# Autodesk Inventor assembly: Tensioner
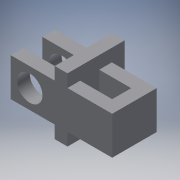
[picture p0: Inventor's stored thumbnail of the model, 180x180]
Saved by Autodesk Inventor 2017 (Build 210142000, 142)
## iProperties
Created: 2017-07-29
Part Number: Tensioner
Document SubType Name: Assembly
Designer: User
Author: User
## Documents named in this file (3)
- C:\Robotics\CAD\2016-17_CAD\DriveTrain\Tensioner.iam
- C:\Robotics\CAD\2016-17_CAD\DriveTrain\TensionerAxleHolder.ipt
- C:\Robotics\CAD\2016-17_CAD\DriveTrain\TensionerPlate.ipt
## Components (2 placed, 2 different names)
1. TensionerAxleHolder:1 — Mate:1, Flush:1
2. TensionerPlate:1 — Mate:1, Flush:1
## Relationships (2: Mate 1, Flush 1)
- Mate:1: TensionerAxleHolder:1 ↔ TensionerPlate:1
- Flush:1 (6.35 mm): TensionerAxleHolder:1 ↔ TensionerPlate:1
